# Autodesk Inventor assembly: Toaster with improved heating elements
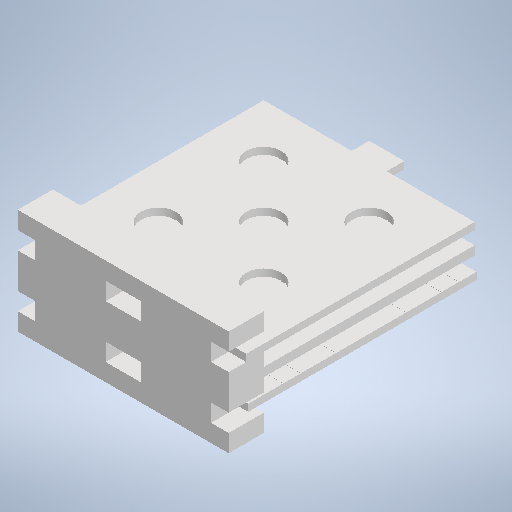
[picture p0: Inventor's stored thumbnail of the model, 512x512]
Saved by Autodesk Inventor 2025.1 (Build 291241020, 241B)
## iProperties
Created: 2024-10-29
Part Number: Toaster with improved heating elements
Document SubType Name: Assembly
Designer: jjk
Author: jjk
## Documents named in this file (5)
- C:\Users\jjk\Desktop\Capstone CAD\Version 3\Toaster with improved heating elements.iam
- C:\Users\jjk\Desktop\Capstone CAD\Version 3\Base.ipt
- C:\Users\jjk\Desktop\Capstone CAD\Version 3\air layer.ipt
- C:\Users\jjk\Desktop\Capstone CAD\Version 3\bread.ipt
- C:\Users\jjk\Desktop\Capstone CAD\Version 3\improved heating plate with heating elements.iam
## Components (6 placed, 4 different names)
1. Base:1 — Mate:5, Flush:7, Mate:7, Mate:9, Mate:11, Mate:12, Mate:13, Mate:14, Flush:10
2. air layer:1 — Mate:5, Flush:7
3. air layer:2 — Mate:7, Flush:9, Mate:10
4. bread:1 — Mate:9, Flush:9, Mate:10
5. improved heating plate with heating elements:1 [sub-assembly] — Mate:13, Mate:14, Flush:10
6. improved heating plate with heating elements:2 [sub-assembly] — Mate:11, Mate:12
## Relationships (11: Mate 8, Flush 3)
- Mate:5: Base:1 ↔ air layer:1
- Flush:7: Base:1 ↔ air layer:1
- Mate:7: Base:1 ↔ air layer:2
- Mate:9: Base:1 ↔ bread:1
- Flush:9: air layer:2 ↔ bread:1
- Mate:10: air layer:2 ↔ bread:1
- Mate:11: Base:1 ↔ improved heating plate with heating elements:2
- Mate:12: Base:1 ↔ improved heating plate with heating elements:2
- Mate:13: Base:1 ↔ improved heating plate with heating elements:1
- Mate:14: Base:1 ↔ improved heating plate with heating elements:1
- Flush:10: Base:1 ↔ improved heating plate with heating elements:1
